# Autodesk Inventor assembly: House_Test
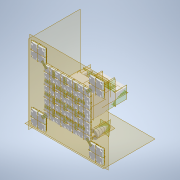
[picture p0: Inventor's stored thumbnail of the model, 180x180]
Saved by Autodesk Inventor 2022.4 (Build 264492010, 492A)
## iProperties
Created: 2025-02-20
Part Number: House_Test
Document SubType Name: Assembly
Designer: jan-m
Author: jan-m
## Documents named in this file (18)
- C:\School\Masterproef\3D Modellen\House_Test.iam
- C:\School\Masterproef\3D Modellen\Tile.ipt
- C:\School\Masterproef\3D Modellen\Tile_Connector.ipt
- C:\School\Masterproef\3D Modellen\Wall.ipt
- C:\School\Masterproef\3D Modellen\Roof_Wall_Small_Left.ipt
- C:\School\Masterproef\3D Modellen\Roof_Wall_Small_Right.ipt
- C:\School\Masterproef\3D Modellen\Roof_Wall_Large_Left.ipt
- C:\School\Masterproef\3D Modellen\Roof_Wall_Large_Right.ipt
- C:\School\Masterproef\3D Modellen\Roof_Small.ipt
- C:\School\Masterproef\3D Modellen\Roof_Large.ipt
- C:\School\Masterproef\3D Modellen\Hanging_Wall.ipt
- C:\School\Masterproef\3D Modellen\1x1_Piece.ipt
- C:\School\Masterproef\3D Modellen\Marker_Tile.ipt
- C:\School\Masterproef\3D Modellen\Tile_Cover.ipt
- C:\School\Masterproef\3D Modellen\Tree_Leaves.ipt
- C:\School\Masterproef\3D Modellen\Tree_Trunk.ipt
- C:\School\Masterproef\3D Modellen\Chimney.ipt
- C:\School\Masterproef\3D Modellen\Pin.ipt
## Components (395 placed, 17 different names)
1. Wall:1 — Mate:10, Mate:11, Mate:12, Mate:40, Mate:46, Mate:59
2. Wall:2 — Mate:13, Mate:14, Mate:15, Mate:27, Mate:28, Mate:30, Mate:31, Mate:60, Mate:64, Mate:72
3. Wall:3 — Mate:19, Mate:20, Mate:21, Mate:37, Mate:42, Mate:58
4. Wall:4 — Mate:16, Mate:17, Mate:18, Mate:23, Mate:25, Mate:33, Mate:34, Mate:63, Mate:65
5. Roof_Wall_Small_Left:2 — Mate:23, Mate:25, Mate:65, Mate:80, Mate:81, Flush:6
6. Roof_Wall_Small_Right:2 — Mate:27, Mate:28, Mate:64, Mate:72
7. Roof_Wall_Large_Left:1 — Mate:30, Mate:31, Mate:60
8. Roof_Wall_Large_Right:1 — Mate:33, Mate:34, Mate:63
9. Roof_Small:1 — Mate:37, Mate:42, Mate:58
10. Roof_Large:1 — Mate:40, Mate:43, Mate:44, Mate:46, Mate:59, Flush:7
11. Hanging_Wall:1 — Mate:43, Mate:44, Flush:7
12. Tree_Leaves:1 — Mate:73, Mate:74
13. Tree_Trunk:1 — Mate:73, Mate:74, Mate:75, Mate:76, Mate:77
14. Chimney:1 — Mate:78, Mate:79, Mate:81, Flush:6
15. Pin:1 — Mate:78, Mate:79, Mate:80
16. Tile_Connector:2 — Mate:6, Mate:7
17. Tile:1 — Mate:2, Mate:5, Mate:6, Mate:7, Mate:16, Mate:91, Mate:92, Mate:96, Mate:97, Mate:98
18. Tile_Connector:1 — Mate:2, Mate:5
19. Tile_Connector:3
20. Tile:2 — Mate:10, Mate:12
21. Tile_Connector:4
22. Tile_Connector:5
23. Tile:3 — Mate:11
24. Tile_Connector:6
25. Tile_Connector:7
26. Tile:4 — Mate:13, Mate:75, Mate:76, Mate:77, Mate:94, Mate:95, Flush:11
27. Tile_Connector:8
28. Tile_Connector:9
29. Tile:5
30. Tile_Connector:10
31. Tile_Connector:11
32. Tile:6
33. Tile_Connector:12
34. Tile_Connector:13
35. Tile:7
36. Tile_Connector:14
37. Tile_Connector:15
38. Tile:8 — Mate:15
39. Tile_Connector:16
40. Tile_Connector:17
41. Tile:9 — Mate:17, Mate:18, Mate:83, Mate:84, Flush:10, Mate:85, Mate:86
42. Tile_Connector:18
43. Tile_Connector:19
44. Tile:10 — Mate:19, Mate:21
45. Tile_Connector:20
46. Tile_Connector:21
47. Tile:11 — Mate:20
48. Tile_Connector:22
49. Tile_Connector:23
50. Tile:12 — Mate:14, Mate:88, Mate:89
51. Tile_Connector:24
52. Tile_Connector:25
53. Tile:13 — Mate:57, Mate:61, Mate:62
54. Tile_Connector:26
55. Tile_Connector:27
56. Tile:14
57. Tile_Connector:28
58. Tile_Connector:29
59. Tile:15
60. Tile_Connector:30
61. Tile_Connector:31
62. Tile:16
63. Tile_Connector:32
64. Tile_Cover:1 — Mate:57, Mate:61, Mate:62
65. Tile_Cover:2
66. Tile_Cover:3
67. Tile_Cover:4
68. 1x1_Piece:147 — Mate:83, Mate:84, Flush:10
69. 1x1_Piece:155
70. 1x1_Piece:156
71. 1x1_Piece:157 — Mate:87
72. 1x1_Piece:158
73. 1x1_Piece:159
74. 1x1_Piece:160
75. 1x1_Piece:161
76. 1x1_Piece:162
77. 1x1_Piece:163
78. 1x1_Piece:164
79. 1x1_Piece:165
80. 1x1_Piece:166
81. 1x1_Piece:167
82. 1x1_Piece:168
83. 1x1_Piece:169
84. 1x1_Piece:170
85. 1x1_Piece:171
86. 1x1_Piece:172
87. 1x1_Piece:173
88. 1x1_Piece:174
89. 1x1_Piece:175
90. 1x1_Piece:176
91. 1x1_Piece:177
92. 1x1_Piece:178
93. 1x1_Piece:179
94. 1x1_Piece:180
95. 1x1_Piece:181
96. 1x1_Piece:182
97. 1x1_Piece:183
98. 1x1_Piece:184
99. 1x1_Piece:185
100. 1x1_Piece:186
101. 1x1_Piece:187
102. 1x1_Piece:188
103. 1x1_Piece:189
104. 1x1_Piece:190
105. 1x1_Piece:191
106. 1x1_Piece:192
107. 1x1_Piece:193
108. 1x1_Piece:194
109. 1x1_Piece:195
110. 1x1_Piece:196
111. 1x1_Piece:197
112. 1x1_Piece:198
113. 1x1_Piece:199
114. 1x1_Piece:200
115. 1x1_Piece:201 — Mate:93
116. 1x1_Piece:202
117. 1x1_Piece:203
118. 1x1_Piece:204
119. 1x1_Piece:205
120. 1x1_Piece:206
121. 1x1_Piece:207
122. 1x1_Piece:208
123. 1x1_Piece:209
124. 1x1_Piece:210
125. 1x1_Piece:211
126. 1x1_Piece:212
127. 1x1_Piece:213
128. 1x1_Piece:146 — Mate:85, Mate:86, Mate:87
129. 1x1_Piece:214
130. 1x1_Piece:215
131. 1x1_Piece:216
132. 1x1_Piece:217
133. 1x1_Piece:218
134. 1x1_Piece:219
135. 1x1_Piece:220
136. 1x1_Piece:221
137. 1x1_Piece:222
138. 1x1_Piece:223
139. 1x1_Piece:224 — Mate:90
140. 1x1_Piece:151 — Mate:88, Mate:89, Mate:90
141. 1x1_Piece:225
142. 1x1_Piece:226
143. 1x1_Piece:227
144. 1x1_Piece:228
145. 1x1_Piece:229
146. 1x1_Piece:230
147. 1x1_Piece:231
148. 1x1_Piece:232
149. 1x1_Piece:233
150. 1x1_Piece:234
151. 1x1_Piece:235
152. 1x1_Piece:236
153. 1x1_Piece:237
154. 1x1_Piece:238
155. 1x1_Piece:239
156. 1x1_Piece:240
157. 1x1_Piece:241
158. 1x1_Piece:242
159. 1x1_Piece:243
160. 1x1_Piece:244
161. 1x1_Piece:245
162. 1x1_Piece:246
163. 1x1_Piece:247
164. 1x1_Piece:248
165. 1x1_Piece:249
166. 1x1_Piece:250
167. 1x1_Piece:251
168. 1x1_Piece:252
169. 1x1_Piece:253
170. 1x1_Piece:254
171. 1x1_Piece:255
172. 1x1_Piece:256
173. 1x1_Piece:257
174. 1x1_Piece:258
175. 1x1_Piece:259
176. 1x1_Piece:260
177. 1x1_Piece:261
178. 1x1_Piece:262
179. 1x1_Piece:263
180. 1x1_Piece:264
181. 1x1_Piece:265
182. 1x1_Piece:266
183. 1x1_Piece:267
184. 1x1_Piece:268
185. 1x1_Piece:269
186. 1x1_Piece:270
187. 1x1_Piece:271
188. 1x1_Piece:272
189. 1x1_Piece:273
190. 1x1_Piece:274
191. 1x1_Piece:275
192. 1x1_Piece:145 — Mate:91, Mate:92, Mate:93
193. 1x1_Piece:276
194. 1x1_Piece:277
195. 1x1_Piece:278
196. 1x1_Piece:279
197. 1x1_Piece:280
198. 1x1_Piece:281
199. 1x1_Piece:282
200. 1x1_Piece:283
201. 1x1_Piece:284
202. 1x1_Piece:285
203. 1x1_Piece:286
204. 1x1_Piece:287
205. 1x1_Piece:288
206. 1x1_Piece:289
207. 1x1_Piece:290
208. 1x1_Piece:291
209. 1x1_Piece:292
210. 1x1_Piece:293
211. 1x1_Piece:294
212. 1x1_Piece:295
213. 1x1_Piece:296
214. 1x1_Piece:297
215. 1x1_Piece:298
216. 1x1_Piece:299
217. 1x1_Piece:300
218. 1x1_Piece:301
219. 1x1_Piece:302
220. 1x1_Piece:303
221. 1x1_Piece:304
222. 1x1_Piece:305
223. 1x1_Piece:306
224. 1x1_Piece:307
225. 1x1_Piece:308
226. 1x1_Piece:309
227. 1x1_Piece:310
228. 1x1_Piece:311
229. 1x1_Piece:312
230. 1x1_Piece:313
231. 1x1_Piece:314
232. 1x1_Piece:315
233. 1x1_Piece:316
234. 1x1_Piece:317
235. 1x1_Piece:318
236. 1x1_Piece:319
237. 1x1_Piece:320
238. 1x1_Piece:321
239. 1x1_Piece:322
240. 1x1_Piece:148 — Mate:94, Mate:95, Flush:11
241. 1x1_Piece:323
242. 1x1_Piece:324
243. 1x1_Piece:325
244. Tile_Connector:33 — Mate:67, Mate:69, Mate:71, Mate:96, Mate:97, Mate:98
245. Marker_Tile:1 — Mate:53, Mate:54, Flush:5, Mate:67, Mate:69, Mate:71, Mate:100, Mate:101
246. Tile_Connector:34
247. Marker_Tile:2
248. Tile_Connector:35
249. Marker_Tile:3
250. Tile_Connector:36
251. Marker_Tile:4
252. 1x1_Piece:1 — Mate:53, Mate:54, Flush:5, Mate:99
253. 1x1_Piece:2
254. 1x1_Piece:3
255. 1x1_Piece:4
256. 1x1_Piece:5
257. 1x1_Piece:6
258. 1x1_Piece:7
259. 1x1_Piece:8
260. 1x1_Piece:9
261. 1x1_Piece:10
262. 1x1_Piece:11
263. 1x1_Piece:12
264. 1x1_Piece:13
265. 1x1_Piece:14
266. 1x1_Piece:15
267. 1x1_Piece:16
268. 1x1_Piece:17
269. 1x1_Piece:18
270. 1x1_Piece:19
271. 1x1_Piece:20
272. 1x1_Piece:21
273. 1x1_Piece:22
274. 1x1_Piece:23
275. 1x1_Piece:24
276. 1x1_Piece:25
277. 1x1_Piece:26
278. 1x1_Piece:27
279. 1x1_Piece:28
280. 1x1_Piece:29
281. 1x1_Piece:30
282. 1x1_Piece:31
283. 1x1_Piece:32
284. 1x1_Piece:33
285. 1x1_Piece:34
286. 1x1_Piece:35
287. 1x1_Piece:36
288. 1x1_Piece:326
289. 1x1_Piece:327
290. 1x1_Piece:328
291. 1x1_Piece:329
292. 1x1_Piece:330
293. 1x1_Piece:331
294. 1x1_Piece:332
295. 1x1_Piece:333
296. 1x1_Piece:334
297. 1x1_Piece:335
298. 1x1_Piece:336
299. 1x1_Piece:337
300. 1x1_Piece:338
301. 1x1_Piece:339
302. 1x1_Piece:340
303. 1x1_Piece:341
304. 1x1_Piece:342
305. 1x1_Piece:343
306. 1x1_Piece:344
307. 1x1_Piece:345
308. 1x1_Piece:346
309. 1x1_Piece:347
310. 1x1_Piece:348
311. 1x1_Piece:349
312. 1x1_Piece:350
313. 1x1_Piece:351
314. 1x1_Piece:352
315. 1x1_Piece:353
316. 1x1_Piece:354
317. 1x1_Piece:355
318. 1x1_Piece:356
319. 1x1_Piece:357
320. 1x1_Piece:358
321. 1x1_Piece:359
322. 1x1_Piece:360
323. 1x1_Piece:361
324. 1x1_Piece:362
325. 1x1_Piece:363
326. 1x1_Piece:364
327. 1x1_Piece:365
328. 1x1_Piece:366
329. 1x1_Piece:367
330. 1x1_Piece:368
331. 1x1_Piece:369
332. 1x1_Piece:370
333. 1x1_Piece:371
334. 1x1_Piece:372
335. 1x1_Piece:373
336. 1x1_Piece:374
337. 1x1_Piece:375
338. 1x1_Piece:376
339. 1x1_Piece:377
340. 1x1_Piece:378
341. 1x1_Piece:379
342. 1x1_Piece:380
343. 1x1_Piece:381
344. 1x1_Piece:382
345. 1x1_Piece:383
346. 1x1_Piece:384
347. 1x1_Piece:385
348. 1x1_Piece:386
349. 1x1_Piece:387
350. 1x1_Piece:388
351. 1x1_Piece:389
352. 1x1_Piece:390
353. 1x1_Piece:391
354. 1x1_Piece:392
355. 1x1_Piece:393
356. 1x1_Piece:394
357. 1x1_Piece:395
358. 1x1_Piece:396
359. 1x1_Piece:397
360. 1x1_Piece:398
361. 1x1_Piece:399
362. 1x1_Piece:400
363. 1x1_Piece:401
364. 1x1_Piece:402
365. 1x1_Piece:403
366. 1x1_Piece:404
367. 1x1_Piece:405
368. 1x1_Piece:406
369. 1x1_Piece:407
370. 1x1_Piece:408
371. 1x1_Piece:409
372. 1x1_Piece:410
373. 1x1_Piece:411
374. 1x1_Piece:412
375. 1x1_Piece:413
376. 1x1_Piece:414
377. 1x1_Piece:415
378. 1x1_Piece:416
379. 1x1_Piece:417
380. 1x1_Piece:418
381. 1x1_Piece:419
382. 1x1_Piece:420
383. 1x1_Piece:421
384. 1x1_Piece:422
385. 1x1_Piece:423
386. 1x1_Piece:424
387. 1x1_Piece:425
388. 1x1_Piece:426
389. 1x1_Piece:427
390. 1x1_Piece:428
391. 1x1_Piece:429
392. 1x1_Piece:430
393. 1x1_Piece:431
394. 1x1_Piece:432
395. 1x1_Piece:433
## Component patterns: (16 elements, first: Tile_Connector:2 + Tile:1 + Tile_Connector:1), (4 elements, first: Tile_Cover:1), (60 elements, first: 1x1_Piece:147), (12 elements, first: 1x1_Piece:146), (52 elements, first: 1x1_Piece:151), (48 elements, first: 1x1_Piece:145), (4 elements, first: 1x1_Piece:148), (4 elements, first: Tile_Connector:33 + Marker_Tile:1), (36 elements, first: 1x1_Piece:1), Component Pattern 2:2 (36 elements), Component Pattern 2:3 (36 elements), Component Pattern 2:4 (36 elements)
## Relationships (78: Mate 73, Flush 5)
- Mate:2: Tile:1 ↔ Tile_Connector:1
- Mate:5: Tile:1 ↔ Tile_Connector:1
- Mate:6: Tile_Connector:2 ↔ Tile:1
- Mate:7: Tile_Connector:2 ↔ Tile:1
- Mate:10: Wall:1 ↔ Tile:2
- Mate:11: Wall:1 ↔ Tile:3
- Mate:12: Wall:1 ↔ Tile:2
- Mate:13: Wall:2 ↔ Tile:4
- Mate:14: Wall:2 ↔ Tile:12
- Mate:15: Wall:2 ↔ Tile:8
- Mate:16: Wall:4 ↔ Tile:1
- Mate:17: Wall:4 ↔ Tile:9
- Mate:18: Wall:4 ↔ Tile:9
- Mate:19: Wall:3 ↔ Tile:10
- Mate:20: Wall:3 ↔ Tile:11
- Mate:21: Wall:3 ↔ Tile:10
- Mate:23: Wall:4 ↔ Roof_Wall_Small_Left:2
- Mate:25: Wall:4 ↔ Roof_Wall_Small_Left:2
- Mate:27: Wall:2 ↔ Roof_Wall_Small_Right:2
- Mate:28: Wall:2 ↔ Roof_Wall_Small_Right:2
- Mate:30: Wall:2 ↔ Roof_Wall_Large_Left:1
- Mate:31: Wall:2 ↔ Roof_Wall_Large_Left:1
- Mate:33: Wall:4 ↔ Roof_Wall_Large_Right:1
- Mate:34: Wall:4 ↔ Roof_Wall_Large_Right:1
- Mate:37: Wall:3 ↔ Roof_Small:1
- Mate:40: Wall:1 ↔ Roof_Large:1
- Mate:42: Wall:3 ↔ Roof_Small:1
- Mate:43: Roof_Large:1 ↔ Hanging_Wall:1
- Mate:44: Roof_Large:1 ↔ Hanging_Wall:1
- Mate:46: Wall:1 ↔ Roof_Large:1
- Mate:53: Marker_Tile:1 ↔ 1x1_Piece:1
- Mate:54: Marker_Tile:1 ↔ 1x1_Piece:1
- Mate:57: Tile:13 ↔ Tile_Cover:1
- Mate:58: Wall:3 ↔ Roof_Small:1
- Mate:59: Wall:1 ↔ Roof_Large:1
- Flush:5: Marker_Tile:1 ↔ 1x1_Piece:1
- Mate:60: Wall:2 ↔ Roof_Wall_Large_Left:1
- Mate:61: Tile:13 ↔ Tile_Cover:1
- Mate:62: Tile:13 ↔ Tile_Cover:1
- Mate:63: Wall:4 ↔ Roof_Wall_Large_Right:1
- Mate:64: Wall:2 ↔ Roof_Wall_Small_Right:2
- Mate:65: Wall:4 ↔ Roof_Wall_Small_Left:2
- Mate:67: Tile_Connector:33 ↔ Marker_Tile:1
- Mate:69: Tile_Connector:33 ↔ Marker_Tile:1
- Mate:71: Tile_Connector:33 ↔ Marker_Tile:1
- Mate:72: Wall:2 ↔ Roof_Wall_Small_Right:2
- Mate:73: Tree_Leaves:1 ↔ Tree_Trunk:1
- Mate:74: Tree_Leaves:1 ↔ Tree_Trunk:1
- Mate:75: Tree_Trunk:1 ↔ Tile:4
- Mate:76: Tree_Trunk:1 ↔ Tile:4
- Mate:77: Tree_Trunk:1 ↔ Tile:4
- Mate:78: Chimney:1 ↔ Pin:1
- Mate:79: Chimney:1 ↔ Pin:1
- Mate:80: Roof_Wall_Small_Left:2 ↔ Pin:1
- Mate:81: Roof_Wall_Small_Left:2 ↔ Chimney:1
- Flush:6: Roof_Wall_Small_Left:2 ↔ Chimney:1
- Flush:7: Roof_Large:1 ↔ Hanging_Wall:1
- Mate:83: Tile:9 ↔ 1x1_Piece:147
- Mate:84: Tile:9 ↔ 1x1_Piece:147
- Flush:10: Tile:9 ↔ 1x1_Piece:147
- Mate:85: Tile:9 ↔ 1x1_Piece:146
- Mate:86: Tile:9 ↔ 1x1_Piece:146
- Mate:87: 1x1_Piece:157 ↔ 1x1_Piece:146
- Mate:88: Tile:12 ↔ 1x1_Piece:151
- Mate:89: Tile:12 ↔ 1x1_Piece:151
- Mate:90: 1x1_Piece:224 ↔ 1x1_Piece:151
- Mate:91: Tile:1 ↔ 1x1_Piece:145
- Mate:92: Tile:1 ↔ 1x1_Piece:145
- Mate:93: 1x1_Piece:201 ↔ 1x1_Piece:145
- Mate:94: Tile:4 ↔ 1x1_Piece:148
- Mate:95: Tile:4 ↔ 1x1_Piece:148
- Flush:11: Tile:4 ↔ 1x1_Piece:148
- Mate:96: Tile:1 ↔ Tile_Connector:33
- Mate:97: Tile:1 ↔ Tile_Connector:33
- Mate:98: Tile:1 ↔ Tile_Connector:33
- Mate:99: 1x1_Piece:1
- Mate:100: Marker_Tile:1
- Mate:101: Marker_Tile:1
